# Autodesk Inventor assembly: kakutome_nc_8
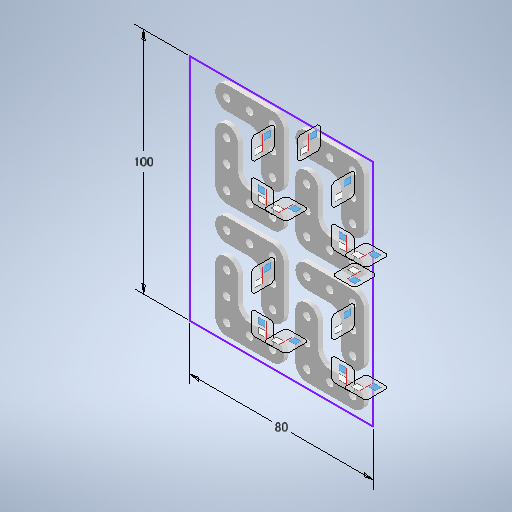
[picture p0: Inventor's stored thumbnail of the model, 512x512]
Saved by Autodesk Inventor 2025.1 (Build 291241000, 241)
## iProperties
Created: 2025-05-05
Part Number: kakutome_nc_8
Document SubType Name: Assembly
Designer: yuki0520
Author: yuki0520
## Documents named in this file (2)
- C:\Users\yuki0520\OneDrive\ドキュメント\Inventor\2025_nhk\tanaka\nageru\smallring\kakutome_nc_8.iam
- C:\Users\yuki0520\OneDrive\ドキュメント\Inventor\2025_nhk\tanaka\nageru\smallring\kakutome_nc.ipt
## Components (8 placed, 1 different names)
1. kakutome_nc:6 — メイト:1, メイト:2, フラッシュ:1, メイト:9, メイト:10
2. kakutome_nc:8 — メイト:1, メイト:2, フラッシュ:1, フラッシュ:5, フラッシュ:6, フラッシュ:7, フラッシュ:10, フラッシュ:11
3. kakutome_nc:9 — メイト:4
4. kakutome_nc:10 — メイト:4, フラッシュ:7, メイト:9, フラッシュ:8, フラッシュ:11
5. kakutome_nc:11 — メイト:6
6. kakutome_nc:12 — メイト:6, フラッシュ:5, メイト:10, フラッシュ:9, フラッシュ:10
7. kakutome_nc:13 — メイト:8
8. kakutome_nc:14 — メイト:8, フラッシュ:6, フラッシュ:8, フラッシュ:9
## Relationships (21: Flush 11, Mate 10)
- メイト:1 [Mate] (10 mm): kakutome_nc:6 ↔ kakutome_nc:8
- メイト:2 [Mate] (25 mm): kakutome_nc:6 ↔ kakutome_nc:8
- フラッシュ:1 [Flush]: kakutome_nc:6 ↔ kakutome_nc:8
- [Mate] (10 mm): kakutome_nc:9 ↔ kakutome_nc:10
- メイト:4 [Mate] (25 mm): kakutome_nc:9 ↔ kakutome_nc:10
- [Flush]: kakutome_nc:9 ↔ kakutome_nc:10
- [Mate] (10 mm): kakutome_nc:11 ↔ kakutome_nc:12
- メイト:6 [Mate] (25 mm): kakutome_nc:11 ↔ kakutome_nc:12
- [Flush]: kakutome_nc:11 ↔ kakutome_nc:12
- [Mate] (10 mm): kakutome_nc:13 ↔ kakutome_nc:14
- メイト:8 [Mate] (25 mm): kakutome_nc:13 ↔ kakutome_nc:14
- [Flush]: kakutome_nc:13 ↔ kakutome_nc:14
- フラッシュ:5 [Flush]: kakutome_nc:8 ↔ kakutome_nc:12
- フラッシュ:6 [Flush]: kakutome_nc:8 ↔ kakutome_nc:14
- フラッシュ:7 [Flush]: kakutome_nc:8 ↔ kakutome_nc:10
- メイト:9 [Mate] (5 mm): kakutome_nc:6 ↔ kakutome_nc:10
- メイト:10 [Mate] (5 mm): kakutome_nc:6 ↔ kakutome_nc:12
- フラッシュ:8 [Flush]: kakutome_nc:10 ↔ kakutome_nc:14
- フラッシュ:9 [Flush]: kakutome_nc:12 ↔ kakutome_nc:14
- フラッシュ:10 [Flush]: kakutome_nc:8 ↔ kakutome_nc:12
- フラッシュ:11 [Flush]: kakutome_nc:8 ↔ kakutome_nc:10
## Named parameters: d44_d41 = 10 mm, d45_d42 = 25 mm, d46_d43 = 0 mm, d47_d41 = 10 mm, d48_d42 = 25 mm, d49_d43 = 0 mm, d50_d41 = 10 mm, d51_d42 = 25 mm, d52_d43 = 0 mm
